# Autodesk Inventor assembly: LEG
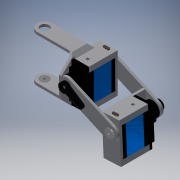
[picture p0: Inventor's stored thumbnail of the model, 180x180]
Saved by Autodesk Inventor 2017 (Build 210142000, 142)
## iProperties
Created: 2017-09-11
Part Number: LEG
Document SubType Name: Assembly
Designer: Alexander Miller
Author: Alexander Miller
## Documents named in this file (6)
- D:\Daten\Documents\Git\HeRo-Mini\Hardware\LEG.iam
- D:\Daten\Documents\Git\HeRo-Mini\Hardware\COXA.ipt
- D:\Daten\Documents\Git\HeRo-Mini\Hardware\SERVO.iam
- D:\Daten\Documents\Git\HeRo-Mini\Hardware\BEARING.ipt
- D:\Daten\Documents\Git\HeRo-Mini\Hardware\FEMUR.ipt
- D:\Daten\Documents\Git\HeRo-Mini\Hardware\TIBIA.ipt
## Components (9 placed, 5 different names)
1. COXA:1 — Rigid:1, Rotational:1, Rotational:3
2. SERVO:1 [sub-assembly] — Rigid:1, Rigid:2
3. BEARING:1 — Rotational:1
4. FEMUR:1 — Rigid:2, Rigid:3
5. FEMUR:2 — Rotational:2, Rigid:5
6. BEARING:2 — Rigid:3
7. BEARING:3 — Rotational:2, Rotational:3
8. TIBIA:1 — Rigid:4
9. SERVO:2 [sub-assembly] — Rigid:4, Rigid:5
## Relationships (8: WeldJoint 5, RevoluteJoint 3)
- Rigid:1 [WeldJoint]: COXA:1 ↔ SERVO:1
- Rotational:1 [RevoluteJoint]: COXA:1 ↔ BEARING:1
- Rigid:2 [WeldJoint]: SERVO:1 ↔ FEMUR:1
- Rigid:3 [WeldJoint]: FEMUR:1 ↔ BEARING:2
- Rotational:2 [RevoluteJoint]: FEMUR:2 ↔ BEARING:3
- Rotational:3 [RevoluteJoint]: COXA:1 ↔ BEARING:3
- Rigid:4 [WeldJoint]: TIBIA:1 ↔ SERVO:2
- Rigid:5 [WeldJoint]: FEMUR:2 ↔ SERVO:2
